# Autodesk Inventor assembly: RPi3_ModelB v1
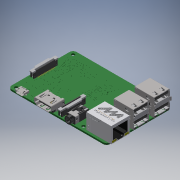
[picture p0: Inventor's stored thumbnail of the model, 180x180]
Saved by Autodesk Inventor 2018 (Build 220112000, 112)
## iProperties
Created: 1999-09-29
Part Number: RPi3_ModelB v1
Document SubType Name: Assembly
Designer: bbramman
Sending System: SolidWorks 2016
Last Author: awillame
Last Saved: 2017-12-17
Author: bbramman
## Documents named in this file (9)
- C:\Users\bbramman\OneDrive\Documents\Trapped Ion Research (Grad)\Electronics\pll-evalboard-synthesizer\Box CAD\RPi3_ModelB v1.iam
- C:\Users\bbramman\OneDrive\Documents\Trapped Ion Research (Grad)\Electronics\pll-evalboard-synthesizer\Box CAD\Rpi components\MOLEX_672983090.ipt
- C:\Users\bbramman\OneDrive\Documents\Trapped Ion Research (Grad)\Electronics\pll-evalboard-synthesizer\Box CAD\Rpi components\molex_0473460001.ipt
- C:\Users\bbramman\OneDrive\Documents\Trapped Ion Research (Grad)\Electronics\pll-evalboard-synthesizer\Box CAD\Rpi components\molex_0471510001.ipt
- C:\Users\bbramman\OneDrive\Documents\Trapped Ion Research (Grad)\Electronics\pll-evalboard-synthesizer\Box CAD\Rpi components\PJ-322.ipt
- C:\Users\bbramman\OneDrive\Documents\Trapped Ion Research (Grad)\Electronics\pll-evalboard-synthesizer\Box CAD\Rpi components\te_1-1734248-5.ipt
- C:\Users\bbramman\OneDrive\Documents\Trapped Ion Research (Grad)\Electronics\pll-evalboard-synthesizer\Box CAD\Rpi components\MOLEX_1040310811.ipt
- C:\Users\bbramman\OneDrive\Documents\Trapped Ion Research (Grad)\Electronics\pll-evalboard-synthesizer\Box CAD\Rpi components\raspberry_pi_B_(RJ45).ipt
- C:\Users\bbramman\OneDrive\Documents\Trapped Ion Research (Grad)\Electronics\pll-evalboard-synthesizer\Box CAD\Raspberry Pi 31.ipt
## Components (10 placed, 8 different names)
1. MOLEX_672983090:1
2. MOLEX_672983090:2
3. molex_0473460001:1
4. molex_0471510001:1
5. PJ-322:1
6. te_1-1734248-5:1
7. te_1-1734248-5:2
8. MOLEX_1040310811:1
9. raspberry_pi_B_(RJ45):1 — Mate:1, Flush:1, Flush:2
10. Raspberry Pi 31:1 — Mate:1, Flush:1, Flush:2
## Relationships (3: Flush 2, Mate 1)
- Mate:1: raspberry_pi_B_(RJ45):1 ↔ Raspberry Pi 31:1
- Flush:1 (2 mm): raspberry_pi_B_(RJ45):1 ↔ Raspberry Pi 31:1
- Flush:2 (-2 mm): raspberry_pi_B_(RJ45):1 ↔ Raspberry Pi 31:1
